# Autodesk Inventor assembly: PlactionWheelwithHubnoBearing
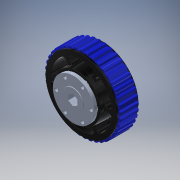
[picture p0: Inventor's stored thumbnail of the model, 180x180]
Saved by Autodesk Inventor 2018 (Build 220112000, 112)
## iProperties
Company: Unknown
Created: 2009-09-26
Part Number: PlactionWheelwithHubnoBearing
Description: Unknown
Document SubType Name: Assembly
Designer: snipe
Sending System: Unknown
Preprocessor: XStep 1.0
Title: //Amserv/amserver/AndyMark/Products/Wheels Solid/Plaction Wheel/4Plaction_500bearing.stp
Author: Unknown
Revision Number: NONE
## Documents named in this file (6)
- E:\Clark\Assets\PlactionWheelwithHubnoBearing.iam
- E:\Clark\Assets\Resources\4MW_d01.ipt
- E:\Clark\Assets\Resources\4RoughTread.ipt
- E:\Clark\Assets\Resources\10-32_nylock_nut.ipt
- E:\Clark\Assets\Resources\10-32x1375_shcs.ipt
- E:\Clark\Assets\500HexHub.ipt
## Components (16 placed, 5 different names)
1. 4MW_d01 — Mate:1, Mate:2, Mate:3
2. 4MW_d01:1
3. 4RoughTread
4. 10-32_nylock_nut
5. 10-32_nylock_nut:1
6. 10-32_nylock_nut:2
7. 10-32_nylock_nut:3
8. 10-32_nylock_nut:4
9. 10-32_nylock_nut:5
10. 10-32x1375_shcs
11. 10-32x1375_shcs:1
12. 10-32x1375_shcs:2
13. 10-32x1375_shcs:3
14. 10-32x1375_shcs:4
15. 10-32x1375_shcs:5
16. 500HexHub:1 — Mate:1, Mate:2, Mate:3
## Relationships (3: Mate 3)
- Mate:1: 4MW_d01 ↔ 500HexHub:1
- Mate:2: 4MW_d01 ↔ 500HexHub:1
- Mate:3: 4MW_d01 ↔ 500HexHub:1
